# Autodesk Inventor assembly: Assembly1
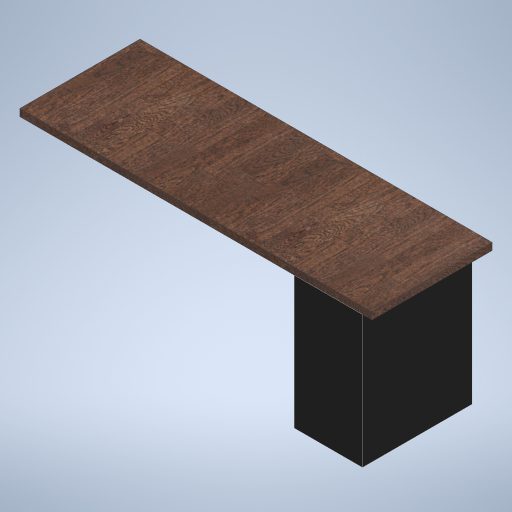
[picture p0: Inventor's stored thumbnail of the model, 512x512]
Saved by Autodesk Inventor 2023 (Build 270158000, 158)
## iProperties
Created: 2023-02-17
Part Number: Assembly1
Document SubType Name: Assembly
Designer: shrey
Author: shrey
## Documents named in this file (8)
- D:\Inventor Projects\headphone cable thing\Assembly1.iam
- D:\Inventor Projects\Wall Vinyl Cover Holder\alex.ipt
- D:\Inventor Projects\headphone cable thing\IKEA KARLBY - walnut, veneer, countertop - 193cm X 65cm.ipt
- D:\Inventor Projects\Wall Vinyl Cover Holder\cord roller.ipt
- D:\Inventor Projects\Wall Vinyl Cover Holder\cord roller housing.ipt
- D:\Inventor Projects\Wall Vinyl Cover Holder\bearing.ipt
- D:\Inventor Projects\Wall Vinyl Cover Holder\bearing cable track.ipt
- D:\Inventor Projects\headphone cable thing\ALEX_Drawer_Unit.dwg
## Components (6 placed, 6 different names)
1. alex:1 — Mate:2, Mate:3, Flush:1, Mate:5, Flush:2, Flush:3, Flush:5, Flush:6, Mate:8, Flush:7, Mate:11, Mate:14
2. IKEA KARLBY - walnut, veneer, countertop - 193cm X 65cm:1 — Mate:5, Flush:2, Flush:3
3. cord roller plate:1 — Mate:7, Flush:4, Flush:5, Flush:6, Flush:8, Flush:10
4. cord roller housing:1 — Mate:8, Mate:9, Mate:10, Flush:7
5. bearing:1 — Mate:11, Mate:12, Mate:13, Flush:8, Mate:17
6. bearing cable track:1 — Mate:14, Mate:15, Mate:16, Flush:10, Mate:17
## Relationships (27: Mate 16, Flush 9, Angle 2)
- Mate:1
- Angle:1 (0 deg)
- Angle:2 (0 deg)
- Mate:2: alex:1
- Mate:3: alex:1
- Flush:1: alex:1
- Mate:4
- Mate:5: alex:1 ↔ IKEA KARLBY - walnut, veneer, countertop - 193cm X 65cm:1
- Flush:2: alex:1 ↔ IKEA KARLBY - walnut, veneer, countertop - 193cm X 65cm:1
- Flush:3 (-50 mm): alex:1 ↔ IKEA KARLBY - walnut, veneer, countertop - 193cm X 65cm:1
- Mate:7: cord roller plate:1
- Flush:4: cord roller plate:1
- Flush:5: alex:1 ↔ cord roller plate:1
- Flush:6: alex:1 ↔ cord roller plate:1
- Mate:8: alex:1 ↔ cord roller housing:1
- Mate:9: cord roller housing:1
- Mate:10: cord roller housing:1
- Flush:7: alex:1 ↔ cord roller housing:1
- Mate:11: alex:1 ↔ bearing:1
- Mate:12: bearing:1
- Mate:13: bearing:1
- Flush:8: cord roller plate:1 ↔ bearing:1
- Mate:14: alex:1 ↔ bearing cable track:1
- Mate:15: bearing cable track:1
- Mate:16: bearing cable track:1
- Flush:10 (-17.25 mm): cord roller plate:1 ↔ bearing cable track:1
- Mate:17: bearing:1 ↔ bearing cable track:1
